# Autodesk Inventor assembly: 12mmsmoothrod_CPY_MIR
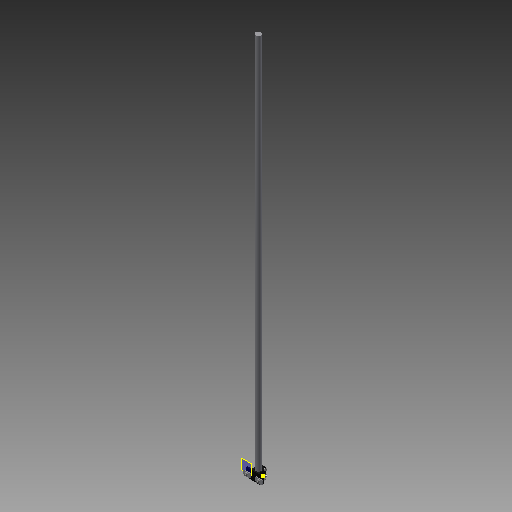
[picture p0: Inventor's stored thumbnail of the model, 512x512]
Saved by Autodesk Inventor 2017 (Build 210142000, 142)
## iProperties
Created: 2016-07-25
Part Number: 12mmsmoothrod_CPY_MIR
Document SubType Name: Assembly
Designer: User
Author: User
## Documents named in this file (7)
- C:\All INVENTOR\SL-Inventor\SL-Beast 3D Printer\12mmsmoothrod_CPY_MIR.iam
- C:\All INVENTOR\SL-Inventor\SL-Beast 3D Printer\12mmSmoothRod_CPY_MIR.ipt
- C:\All INVENTOR\SL-Inventor\SL-Beast 3D Printer\12mmrodholder_CPY_MIR.ipt
- C:\All INVENTOR\SL-Inventor\SL-Beast 3D Printer\en-US\ANSI B18.3.1M(6)\ANSI B18.3.1M - M5x0.8 x 10(1).ipt
- C:\All INVENTOR\SL-Inventor\SL-Beast 3D Printer\M5 Tee Nut-Generic_MIR_CPY_CPY_MIR.ipt
- C:\All INVENTOR\SL-Inventor\SL-Beast 3D Printer\en-US\ANSI B18.3.1M(6)\ANSI B18.3.1M - M3x0.5 x 10(1).ipt
- C:\All INVENTOR\SL-Inventor\SL-Beast 3D Printer\en-US\ANSI B18.16.3M(2)\ANSI B18.16.3M - Property Class 5 and 10 - Metric M3 x 0.5 Metal Type.ipt
## Components (34 placed, 6 different names)
1. 12mmSmoothRod_CPY_MIR:1 — Mate:1
2. 12mmrodholder_CPY_MIR:1 — Mate:1, Insert:1, Insert:2, Insert:3, Insert:4, Insert:5, Insert:6, Insert:7, Insert:8, Insert:9, Insert:10, Insert:11, Insert:12, Insert:13, Insert:14, Insert:15, Insert:16, Insert:17, Insert:18, Insert:19, Insert:20, Insert:21, Insert:22, Insert:23, Insert:24, Insert:25, Insert:26, Insert:27, Insert:28, Mate:5, Mate:7
3. Forged Socket Head Cap Screw - Metric M5x0.8 x 10:1 — Insert:1, Mate:2
4. Forged Socket Head Cap Screw - Metric M5x0.8 x 10:2 — Insert:2, Mate:3
5. M5 Tee Nut-Generic_MIR_CPY_CPY_MIR:1 — Mate:2, Flush:1
6. M5 Tee Nut-Generic_MIR_CPY_CPY_MIR:2 — Flush:1, Mate:3
7. Forged Socket Head Cap Screw - Metric M3x0.5 x 10:1 — Insert:3, Mate:4
8. Forged Socket Head Cap Screw - Metric M3x0.5 x 10:2 — Insert:4
9. Forged Socket Head Cap Screw - Metric M3x0.5 x 10:3 — Insert:5
10. Forged Socket Head Cap Screw - Metric M3x0.5 x 10:4 — Insert:6
11. Forged Socket Head Cap Screw - Metric M3x0.5 x 10:5 — Insert:7
12. Forged Socket Head Cap Screw - Metric M3x0.5 x 10:6 — Insert:8
13. Forged Socket Head Cap Screw - Metric M3x0.5 x 10:7 — Insert:9
14. Forged Socket Head Cap Screw - Metric M3x0.5 x 10:8 — Insert:10
15. Forged Socket Head Cap Screw - Metric M3x0.5 x 10:9 — Insert:11
16. Forged Socket Head Cap Screw - Metric M3x0.5 x 10:10 — Insert:12
17. Forged Socket Head Cap Screw - Metric M3x0.5 x 10:11 — Insert:13
18. Forged Socket Head Cap Screw - Metric M3x0.5 x 10:12 — Insert:14
19. Forged Socket Head Cap Screw - Metric M3x0.5 x 10:13 — Insert:15
20. Forged Socket Head Cap Screw - Metric M3x0.5 x 10:14 — Insert:16
21. Forged Socket Head Cap Screw - Metric M3x0.5 x 10:15 — Insert:17
22. Forged Socket Head Cap Screw - Metric M3x0.5 x 10:16 — Insert:18
23. Forged Socket Head Cap Screw - Metric M3x0.5 x 10:17 — Insert:19
24. Forged Socket Head Cap Screw - Metric M3x0.5 x 10:18 — Insert:20
25. Forged Socket Head Cap Screw - Metric M3x0.5 x 10:19 — Insert:21
26. Forged Socket Head Cap Screw - Metric M3x0.5 x 10:20 — Insert:22
27. Forged Socket Head Cap Screw - Metric M3x0.5 x 10:21 — Insert:23
28. Forged Socket Head Cap Screw - Metric M3x0.5 x 10:22 — Insert:24
29. Forged Socket Head Cap Screw - Metric M3x0.5 x 10:23 — Insert:25
30. Forged Socket Head Cap Screw - Metric M3x0.5 x 10:24 — Insert:26
31. Forged Socket Head Cap Screw - Metric M3x0.5 x 10:25 — Insert:27, Mate:6
32. Forged Socket Head Cap Screw - Metric M3x0.5 x 10:26 — Insert:28
33. Prevailing Torque Type Hex Nut - Steel Metric Property Class 5 and 10 - Metric M3 x 0.5 Metal Type:1 — Mate:4, Mate:5
34. Prevailing Torque Type Hex Nut - Steel Metric Property Class 5 and 10 - Metric M3 x 0.5 Metal Type:2 — Mate:6, Mate:7
## Relationships (36: Insert 28, Mate 7, Flush 1)
- Mate:1: 12mmSmoothRod_CPY_MIR:1 ↔ 12mmrodholder_CPY_MIR:1
- Insert:1: 12mmrodholder_CPY_MIR:1 ↔ Forged Socket Head Cap Screw - Metric M5x0.8 x 10:1
- Insert:2: 12mmrodholder_CPY_MIR:1 ↔ Forged Socket Head Cap Screw - Metric M5x0.8 x 10:2
- Mate:2: Forged Socket Head Cap Screw - Metric M5x0.8 x 10:1 ↔ M5 Tee Nut-Generic_MIR_CPY_CPY_MIR:1
- Flush:1: M5 Tee Nut-Generic_MIR_CPY_CPY_MIR:1 ↔ M5 Tee Nut-Generic_MIR_CPY_CPY_MIR:2
- Mate:3: Forged Socket Head Cap Screw - Metric M5x0.8 x 10:2 ↔ M5 Tee Nut-Generic_MIR_CPY_CPY_MIR:2
- Insert:3: 12mmrodholder_CPY_MIR:1 ↔ Forged Socket Head Cap Screw - Metric M3x0.5 x 10:1
- Insert:4: 12mmrodholder_CPY_MIR:1 ↔ Forged Socket Head Cap Screw - Metric M3x0.5 x 10:2
- Insert:5: 12mmrodholder_CPY_MIR:1 ↔ Forged Socket Head Cap Screw - Metric M3x0.5 x 10:3
- Insert:6: 12mmrodholder_CPY_MIR:1 ↔ Forged Socket Head Cap Screw - Metric M3x0.5 x 10:4
- Insert:7: 12mmrodholder_CPY_MIR:1 ↔ Forged Socket Head Cap Screw - Metric M3x0.5 x 10:5
- Insert:8: 12mmrodholder_CPY_MIR:1 ↔ Forged Socket Head Cap Screw - Metric M3x0.5 x 10:6
- Insert:9: 12mmrodholder_CPY_MIR:1 ↔ Forged Socket Head Cap Screw - Metric M3x0.5 x 10:7
- Insert:10: 12mmrodholder_CPY_MIR:1 ↔ Forged Socket Head Cap Screw - Metric M3x0.5 x 10:8
- Insert:11: 12mmrodholder_CPY_MIR:1 ↔ Forged Socket Head Cap Screw - Metric M3x0.5 x 10:9
- Insert:12: 12mmrodholder_CPY_MIR:1 ↔ Forged Socket Head Cap Screw - Metric M3x0.5 x 10:10
- Insert:13: 12mmrodholder_CPY_MIR:1 ↔ Forged Socket Head Cap Screw - Metric M3x0.5 x 10:11
- Insert:14: 12mmrodholder_CPY_MIR:1 ↔ Forged Socket Head Cap Screw - Metric M3x0.5 x 10:12
- Insert:15: 12mmrodholder_CPY_MIR:1 ↔ Forged Socket Head Cap Screw - Metric M3x0.5 x 10:13
- Insert:16: 12mmrodholder_CPY_MIR:1 ↔ Forged Socket Head Cap Screw - Metric M3x0.5 x 10:14
- Insert:17: 12mmrodholder_CPY_MIR:1 ↔ Forged Socket Head Cap Screw - Metric M3x0.5 x 10:15
- Insert:18: 12mmrodholder_CPY_MIR:1 ↔ Forged Socket Head Cap Screw - Metric M3x0.5 x 10:16
- Insert:19: 12mmrodholder_CPY_MIR:1 ↔ Forged Socket Head Cap Screw - Metric M3x0.5 x 10:17
- Insert:20: 12mmrodholder_CPY_MIR:1 ↔ Forged Socket Head Cap Screw - Metric M3x0.5 x 10:18
- Insert:21: 12mmrodholder_CPY_MIR:1 ↔ Forged Socket Head Cap Screw - Metric M3x0.5 x 10:19
- Insert:22: 12mmrodholder_CPY_MIR:1 ↔ Forged Socket Head Cap Screw - Metric M3x0.5 x 10:20
- Insert:23: 12mmrodholder_CPY_MIR:1 ↔ Forged Socket Head Cap Screw - Metric M3x0.5 x 10:21
- Insert:24: 12mmrodholder_CPY_MIR:1 ↔ Forged Socket Head Cap Screw - Metric M3x0.5 x 10:22
- Insert:25: 12mmrodholder_CPY_MIR:1 ↔ Forged Socket Head Cap Screw - Metric M3x0.5 x 10:23
- Insert:26: 12mmrodholder_CPY_MIR:1 ↔ Forged Socket Head Cap Screw - Metric M3x0.5 x 10:24
- Insert:27: 12mmrodholder_CPY_MIR:1 ↔ Forged Socket Head Cap Screw - Metric M3x0.5 x 10:25
- Insert:28: 12mmrodholder_CPY_MIR:1 ↔ Forged Socket Head Cap Screw - Metric M3x0.5 x 10:26
- Mate:4: Forged Socket Head Cap Screw - Metric M3x0.5 x 10:1 ↔ Prevailing Torque Type Hex Nut - Steel Metric Property Class 5 and 10 - Metric M3 x 0.5 Metal Type:1
- Mate:5: 12mmrodholder_CPY_MIR:1 ↔ Prevailing Torque Type Hex Nut - Steel Metric Property Class 5 and 10 - Metric M3 x 0.5 Metal Type:1
- Mate:6: Forged Socket Head Cap Screw - Metric M3x0.5 x 10:25 ↔ Prevailing Torque Type Hex Nut - Steel Metric Property Class 5 and 10 - Metric M3 x 0.5 Metal Type:2
- Mate:7: 12mmrodholder_CPY_MIR:1 ↔ Prevailing Torque Type Hex Nut - Steel Metric Property Class 5 and 10 - Metric M3 x 0.5 Metal Type:2
